# Autodesk Inventor assembly: Elder-Berry
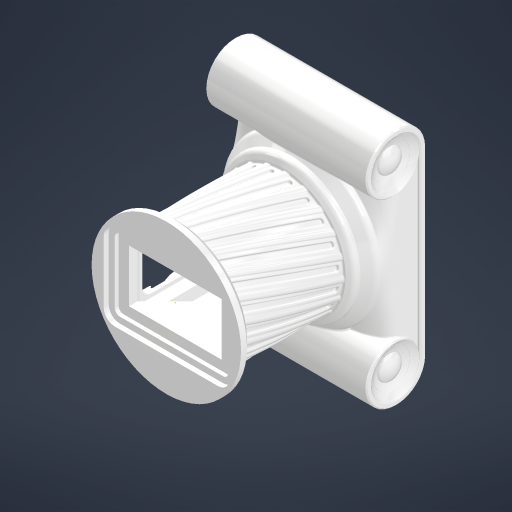
[picture p0: Inventor's stored thumbnail of the model, 512x512]
Saved by Autodesk Inventor 2023 (Build 270158000, 158)
## iProperties
Created: 2026-03-15
Part Number: Elder-Berry
Document SubType Name: Assembly
Designer: lerat
Author: lerat
## Documents named in this file (4)
- C:\Dev\Elder-Berry\hardware\enclosure\Elder-Berry.iam
- C:\Users\lerat\Desktop\top.ipt
- C:\Dev\Elder-Berry\hardware\enclosure\master.ipt
- C:\Dev\Elder-Berry\hardware\enclosure\middle.ipt
## Components (3 placed, 3 different names)
1. top:1 — Einfügen:1
2. master:1 — Einfügen:1
3. middle:1
## Relationships (1: Insert 1)
- Einfügen:1 [Insert]: top:1 ↔ master:1
